# Autodesk Inventor assembly: mirror_assembly_final
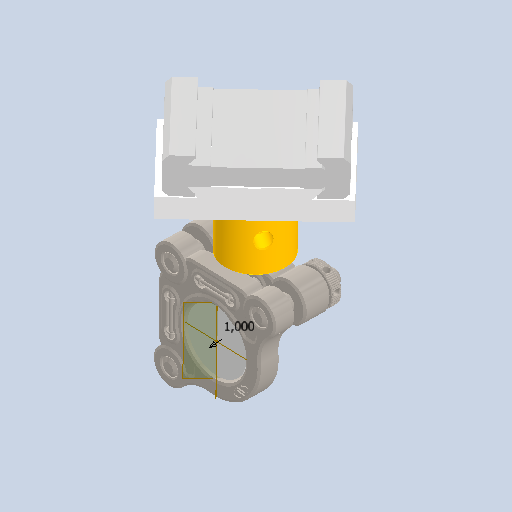
[picture p0: Inventor's stored thumbnail of the model, 512x512]
Saved by Autodesk Inventor 2026.1 (Build 301233000, 233)
## iProperties
Created: 2019-05-24
Part Number: mirror_assembly_final
Document SubType Name: Assembly
Designer: Julian
Author: Julian
## Documents named in this file (6)
- C:\Users\user\Desktop\setup for publishing\mirror_assembly_final.iam
- C:\Users\user\Desktop\setup for publishing\XT66C2-Step_rail mount.ipt
- C:\Users\user\Desktop\setup for publishing\XT66D2-40-Step_post_mount.ipt
- C:\Users\user\Desktop\setup for publishing\M-PS-1E_1in_post.ipt
- C:\Users\user\Desktop\setup for publishing\SS100-F2H_suprema_1in_mirror_mount.ipt
- C:\Users\user\Desktop\setup for publishing\1in_5mm_Beamsplitter.ipt
## Components (5 placed, 5 different names)
1. XT66C2-Step_rail mount:1 — Mate:5, Mate:6, Flush:1
2. XT66D2-40-Step_post_mount:1 — Mate:3, Mate:4, Mate:5, Mate:6, Flush:1, Angle:1
3. M-PS-1E_1in_post:1 — Mate:1, Mate:2, Mate:3, Mate:4
4. SS100-F2H_suprema_1in_mirror_mount:1 — Mate:1, Mate:2, Mate:7, Mate:8
5. 1in_5mm_Beamsplitter:1 — Mate:7, Mate:8, Angle:1
## Relationships (10: Mate 8, Flush 1, Angle 1)
- Mate:1: M-PS-1E_1in_post:1 ↔ SS100-F2H_suprema_1in_mirror_mount:1
- Mate:2: M-PS-1E_1in_post:1 ↔ SS100-F2H_suprema_1in_mirror_mount:1
- Mate:3: XT66D2-40-Step_post_mount:1 ↔ M-PS-1E_1in_post:1
- Mate:4: XT66D2-40-Step_post_mount:1 ↔ M-PS-1E_1in_post:1
- Mate:5: XT66C2-Step_rail mount:1 ↔ XT66D2-40-Step_post_mount:1
- Mate:6: XT66C2-Step_rail mount:1 ↔ XT66D2-40-Step_post_mount:1
- Flush:1 (-0.0508 mm): XT66C2-Step_rail mount:1 ↔ XT66D2-40-Step_post_mount:1
- Mate:7: SS100-F2H_suprema_1in_mirror_mount:1 ↔ 1in_5mm_Beamsplitter:1
- Mate:8: SS100-F2H_suprema_1in_mirror_mount:1 ↔ 1in_5mm_Beamsplitter:1
- Angle:1 (0 deg): XT66D2-40-Step_post_mount:1 ↔ 1in_5mm_Beamsplitter:1
